# Autodesk Inventor assembly: tibia kiri
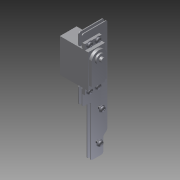
[picture p0: Inventor's stored thumbnail of the model, 180x180]
Saved by Autodesk Inventor 2012 (Build 160160000, 160)
## iProperties
Created: 2013-12-06
Part Number: tibia kiri
Document SubType Name: Assembly
Designer: Irwan Haryanto
Author: Irwan Haryanto
## Documents named in this file (4)
- D:\Revenant\robot baru 2014\tibia kiri.iam
- D:\Revenant\robot baru 2014\riset tibia alumunium 1.ipt
- D:\Revenant\robot baru 2014\servo HS-7955GT.ipt
- D:\Revenant\robot baru 2014\tibia kiri\Design Accelerator\Bolted Connection1.iam
## Components (4 placed, 3 different names)
1. riset tibia alumunium 1:1 — Insert:3, Insert:4, Mate:2
2. riset tibia alumunium 1:2 — Insert:3, Insert:4, Insert:5, Insert:6
3. servo HS-7955GT:1 — Insert:5, Insert:6, Mate:1
4. Bolted Connection:1 [sub-assembly] — Mate:1, Mate:2
## Relationships (6: Insert 4, Mate 2)
- Insert:3 (3 mm): riset tibia alumunium 1:1 ↔ riset tibia alumunium 1:2
- Insert:4 (3 mm): riset tibia alumunium 1:1 ↔ riset tibia alumunium 1:2
- Insert:5: riset tibia alumunium 1:2 ↔ servo HS-7955GT:1
- Insert:6: riset tibia alumunium 1:2 ↔ servo HS-7955GT:1
- Mate:1: servo HS-7955GT:1 ↔ Bolted Connection:1
- Mate:2: riset tibia alumunium 1:1 ↔ Bolted Connection:1
